# Autodesk Inventor assembly: Assembly2
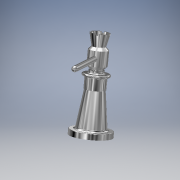
[picture p0: Inventor's stored thumbnail of the model, 180x180]
Saved by Autodesk Inventor 2018 (Build 220112000, 112)
## iProperties
Created: 2019-09-19
Part Number: Assembly2
Document SubType Name: Assembly
Designer: Sameer
Author: Sameer
## Documents named in this file (8)
- C:\Users\Sameer\Desktop\Saad\SMA\Screw Jack\Assembly2.iam
- C:\Users\Sameer\Desktop\Saad\SMA\Screw Jack\Screw jack.ipt
- C:\Users\Sameer\Desktop\Saad\SMA\Screw Jack\Nut of Screw Jack.ipt
- C:\Users\Sameer\Desktop\Saad\SMA\Screw Jack\Spindle.ipt
- C:\Users\Sameer\Desktop\Saad\SMA\Screw Jack\Screw Jack Cup.ipt
- C:\Users\Sameer\Desktop\Saad\SMA\Screw Jack\Washer.ipt
- C:\Users\Sameer\Desktop\Saad\SMA\Screw Jack\Screw.ipt
- C:\Users\Sameer\Desktop\Saad\SMA\Screw Jack\Tommy Bar.ipt
## Components (7 placed, 7 different names)
1. Screw jack:1 — Rigid:1
2. Nut of Screw Jack:1 — Rigid:1, Cylindrical:1
3. Spindle:1 — Cylindrical:1, Rigid:2, Rigid:3, Cylindrical:2, Cylindrical:3
4. Screw Jack Cup:1 — Rigid:2
5. Washer:1 — Rigid:3
6. Screw:1 — Cylindrical:2
7. Tommy Bar:1 — Cylindrical:3
## Relationships (6: WeldJoint 3, CylindricalJoint 3)
- Rigid:1 [WeldJoint]: Screw jack:1 ↔ Nut of Screw Jack:1
- Cylindrical:1: Nut of Screw Jack:1 ↔ Spindle:1
- Rigid:2 [WeldJoint]: Spindle:1 ↔ Screw Jack Cup:1
- Rigid:3 [WeldJoint]: Spindle:1 ↔ Washer:1
- Cylindrical:2: Spindle:1 ↔ Screw:1
- Cylindrical:3: Spindle:1 ↔ Tommy Bar:1
